# Autodesk Inventor assembly: EDMPumpRegionAssembly
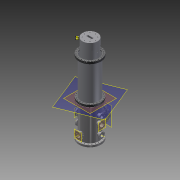
[picture p0: Inventor's stored thumbnail of the model, 180x180]
Saved by Autodesk Inventor 2015 (Build 190159000, 159)
## iProperties
Created: 2014-03-24
Part Number: EDMPumpRegionAssembly
Document SubType Name: Assembly
Designer: jad211
Author: jad211
## Documents named in this file (7)
- C:\CADFiles\EDM New Pumping Region\EDMPumpRegionAssembly.iam
- C:\CADFiles\EDM New Pumping Region\NewHorn.ipt
- C:\CADFiles\EDM New Pumping Region\WG18FLANGECutDown.ipt
- C:\CADFiles\EDM Middle Shield\EDM Middle shield.ipt
- C:\CADFiles\EDM Inner Shield\Inner Shield.iam
- C:\CADFiles\EDM Beamline\Chamber parts\hudson chamber actual size.ipt
- C:\CADFiles\EDM Beamline\Chamber parts\Centre nipple.iam
## Components (7 placed, 6 different names)
1. NewHorn:1 — Flush:10, Mate:1, Mate:2, Mate:4, Mate:6, Flush:12, Mate:11
2. WG18FLANGECutDown:1 — Flush:10, Mate:1, Mate:2, Mate:3, Mate:5
3. WG18FLANGECutDown:2 — Mate:3, Mate:4, Mate:5, Mate:6
4. EDM Middle shield:1 — Mate:8, Flush:11
5. Inner Shield:1 [sub-assembly] — Flush:14, Mate:10, Flush:13
6. hudson chamber actual size:1 — Mate:12, Flush:15, Angle:1, Mate:13
7. Centre nipple:1 [sub-assembly] — Mate:13, Flush:17
## Relationships (24: Mate 12, Flush 11, Angle 1)
- Flush:6 (17 mm)
- Flush:7 (-17 mm)
- Flush:8 (3 mm)
- Flush:10: NewHorn:1 ↔ WG18FLANGECutDown:1
- Mate:1: NewHorn:1 ↔ WG18FLANGECutDown:1
- Mate:2: NewHorn:1 ↔ WG18FLANGECutDown:1
- Mate:3: WG18FLANGECutDown:1 ↔ WG18FLANGECutDown:2
- Mate:4: NewHorn:1 ↔ WG18FLANGECutDown:2
- Mate:5: WG18FLANGECutDown:1 ↔ WG18FLANGECutDown:2
- Mate:6: NewHorn:1 ↔ WG18FLANGECutDown:2
- Mate:8: EDM Middle shield:1
- Flush:11 (158.75 mm): EDM Middle shield:1
- Flush:14 (64.29 mm): Inner Shield:1
- Mate:10: Inner Shield:1
- Flush:12 (-6 mm): NewHorn:1
- Mate:11 (-6 mm): NewHorn:1
- Flush:13: Inner Shield:1
- Mate:12: hudson chamber actual size:1
- Flush:15: hudson chamber actual size:1
- Flush:16 (-304.8 mm)
- Angle:1 (0 deg): hudson chamber actual size:1
- Mate:13: hudson chamber actual size:1 ↔ Centre nipple:1
- Flush:17: Centre nipple:1
- Mate:14
